# Autodesk Inventor assembly: Drivebase
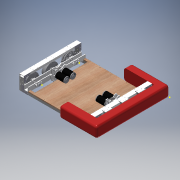
[picture p0: Inventor's stored thumbnail of the model, 180x180]
Saved by Autodesk Inventor 2019 (Build 230136000, 136)
## iProperties
Created: 2018-06-29
Part Number: Drivebase
Document SubType Name: Assembly
Designer: s-2512711
Author: s-2512711
## Documents named in this file (17)
- D:\Summer Drive Base V1\Summer Drivebase\Summer Drivebase.iam
- D:\Summer Drive Base V1\Summer Drivebase\1x1.ipt
- D:\Summer Drive Base V1\Summer Drivebase\pan.ipt
- D:\Summer Drive Base V1\Summer Drivebase\Drivebase PowerUp Files\Gearbox.iam
- D:\Summer Drive Base V1\Summer Drivebase\U.ipt
- D:\Summer Drive Base V1\Summer Drivebase\Drivebase PowerUp Files\Gearbox_CPY.iam
- D:\Summer Drive Base V1\Summer Drivebase\Drivebase PowerUp Files\4461-17-0101 + Bearing.iam
- D:\Summer Drive Base V1\Summer Drivebase\16th hex spacer.ipt
- D:\Summer Drive Base V1\Summer Drivebase\colsonwgeelwithhub.iam
- D:\Summer Drive Base V1\Summer Drivebase\475 hex shaft.ipt
- D:\Summer Drive Base V1\Summer Drivebase\am-1238+Collar+Clamp,+0.5''+Hex+Bore,+Aluminum.iam
- D:\Summer Drive Base V1\Summer Drivebase\Drivebase PowerUp Files\Omni Wheel.iam
- D:\Summer Drive Base V1\Summer Drivebase\525 hex shaft.ipt
- D:\Summer Drive Base V1\Summer Drivebase\5.5 2x2.ipt
- D:\Summer Drive Base V1\Summer Drivebase\26 1x2.ipt
- D:\Summer Drive Base V1\Summer Drivebase\L gusset.ipt
- D:\Summer Drive Base V1\Summer Drivebase\Bumper v2.iam
## Components (65 placed, 16 different names)
1. 1x1:1 — Mate:22, Mate:23, Mate:24, Mate:25, Mate:26, Mate:33, Mate:34, Mate:35, Mate:130, Mate:134
2. 1x1:2 — Mate:48, Mate:49, Mate:50, Mate:128, Mate:136, Mate:137, Mate:169, Mate:170
3. pan:1 — Mate:22, Mate:23, Mate:46, Mate:47
4. Gearbox:1 [sub-assembly] — Mate:36, Mate:37, Mate:42, Rotation:1, Mate:67, Mate:68, Mate:76, Mate:77
5. Gearbox:2 [sub-assembly] — Mate:38, Mate:39, Mate:40, Rotation:2, Mate:70, Mate:71, Mate:73, Mate:74
6. U:1 — Mate:33, Mate:34, Mate:35, Mate:38, Mate:39, Mate:40, Mate:44, Mate:45, Mate:46, Mate:47, Mate:48, Mate:49, Mate:50, Mate:51, Mate:52, Angle:1, Mate:53, Mate:54, Angle:2, Mate:55, Mate:56, Angle:3, Mate:57, Mate:58, Angle:4, Mate:132, Mate:133, Mate:135
7. U:2 — Mate:24, Mate:25, Mate:26, Mate:36, Mate:37, Mate:41, Mate:42, Mate:43, Mate:59, Mate:60, Angle:5, Mate:61, Mate:62, Angle:6, Mate:63, Mate:64, Angle:7, Mate:65, Mate:66, Angle:8, Mate:126, Mate:127, Mate:129, Mate:131, Mate:179
8. Gearbox_CPY:1 [sub-assembly] — Mate:44, Mate:45, Rotation:2, Mate:72
9. Gearbox_CPY:2 [sub-assembly] — Mate:41, Mate:43, Rotation:1, Mate:69
10. 4461-17-0101 + Bearing:1 [sub-assembly] — Mate:55, Mate:56, Angle:3, Mate:98
11. 4461-17-0101 + Bearing:2 [sub-assembly] — Mate:51, Mate:52, Angle:1, Mate:118
12. 4461-17-0101 + Bearing:3 [sub-assembly] — Mate:63, Mate:64, Angle:7, Mate:104, Flush:6, Flush:7
13. 4461-17-0101 + Bearing:4 [sub-assembly] — Mate:59, Mate:60, Angle:5, Mate:79, Mate:80, Mate:81, Rotation:3
14. 4461-17-0101 + Bearing:5 [sub-assembly] — Mate:61, Mate:62, Angle:6, Mate:86
15. 4461-17-0101 + Bearing:6 [sub-assembly] — Mate:65, Mate:66, Angle:8, Mate:109
16. 4461-17-0101 + Bearing:7 [sub-assembly] — Mate:53, Mate:54, Angle:2, Mate:115, Flush:10, Flush:11
17. 4461-17-0101 + Bearing:8 [sub-assembly] — Mate:57, Mate:58, Angle:4, Mate:92, Mate:93, Flush:3
18. 16th hex spacer:1 — Mate:67, Mate:68, Mate:69, Mate:78
19. 16th hex spacer:2 — Mate:70, Mate:71, Mate:72, Mate:75
20. colsonwgeelwithhub:1 [sub-assembly] — Mate:73, Mate:74, Mate:75
21. colsonwgeelwithhub:2 [sub-assembly] — Mate:76, Mate:77, Mate:78
22. 475 hex shaft:1 — Flush:4, Mate:94, Mate:95, Mate:96, Mate:97, Mate:100, Mate:101, Flush:5, Mate:102, Mate:103
23. 475 hex shaft:2 — Mate:82, Mate:83, Flush:1, Mate:84, Mate:85, Mate:87, Mate:88, Mate:90, Mate:91, Flush:2
24. am-1238+Collar+Clamp,+0.5''+Hex+Bore,+Aluminum:1 [sub-assembly] — Mate:92, Mate:93, Flush:3, Flush:4, Mate:94, Mate:95
25. am-1238+Collar+Clamp,+0.5''+Hex+Bore,+Aluminum:2 [sub-assembly] — Mate:79, Mate:80, Mate:81, Rotation:3, Mate:82, Mate:83, Flush:1
26. am-1238+Collar+Clamp,+0.5''+Hex+Bore,+Aluminum:3 [sub-assembly] — Mate:90, Mate:91, Flush:2
27. am-1238+Collar+Clamp,+0.5''+Hex+Bore,+Aluminum:4 [sub-assembly] — Flush:5, Mate:102, Mate:103
28. Omni Wheel:1 [sub-assembly] — Mate:87, Mate:88, Mate:89
29. Omni Wheel:2 [sub-assembly] — Mate:99, Mate:100, Mate:101
30. 16th hex spacer:3 — Mate:84, Mate:85, Mate:86, Mate:89
31. 16th hex spacer:4 — Mate:96, Mate:97, Mate:98, Mate:99
32. 525 hex shaft:1 — Flush:12, Mate:116, Mate:117, Mate:119, Mate:120, Mate:122, Mate:123, Flush:13, Mate:124, Mate:125
33. 525 hex shaft:2 — Flush:8, Mate:105, Mate:106, Mate:107, Mate:108, Mate:110, Mate:111, Mate:113, Mate:114, Flush:9
34. am-1238+Collar+Clamp,+0.5''+Hex+Bore,+Aluminum:5 [sub-assembly] — Mate:115, Flush:10, Flush:11, Flush:12, Mate:116, Mate:117
35. am-1238+Collar+Clamp,+0.5''+Hex+Bore,+Aluminum:6 [sub-assembly] — Mate:104, Flush:6, Flush:7, Flush:8, Mate:105, Mate:106
36. am-1238+Collar+Clamp,+0.5''+Hex+Bore,+Aluminum:7 [sub-assembly] — Flush:13, Mate:124, Mate:125
37. am-1238+Collar+Clamp,+0.5''+Hex+Bore,+Aluminum:8 [sub-assembly] — Mate:113, Mate:114, Flush:9
38. colsonwgeelwithhub:3 [sub-assembly] — Mate:110, Mate:111, Mate:112
39. colsonwgeelwithhub:4 [sub-assembly] — Mate:121, Mate:122, Mate:123
40. 16th hex spacer:5 — Mate:107, Mate:108, Mate:109, Mate:112
41. 16th hex spacer:6 — Mate:118, Mate:119, Mate:120, Mate:121
42. 5.5 2x2:1 — Mate:126, Mate:127, Mate:128, Mate:138, Mate:139, Mate:140, Mate:148, Mate:168, Mate:171, Mate:172, Mate:196
43. 5.5 2x2:2 — Mate:135, Mate:136, Mate:137, Mate:141, Mate:142, Mate:143, Mate:152, Mate:155, Mate:186, Mate:188, Mate:189, Mate:190, Mate:191, Mate:192
44. 5.5 2x2:3 — Mate:132, Mate:133, Mate:134, Mate:180, Mate:182, Mate:183, Mate:184, Mate:193, Mate:194, Mate:198
45. 5.5 2x2:4 — Mate:129, Mate:130, Mate:131, Mate:174, Mate:176, Mate:177, Mate:178, Mate:195
46. 26 1x2:1 — Mate:141, Mate:142, Mate:143, Mate:150, Mate:151, Mate:153, Mate:154, Mate:156, Mate:157, Mate:158, Mate:159, Mate:160, Mate:161, Mate:197, Mate:199
47. 26 1x2:2 — Mate:138, Mate:139, Mate:140, Mate:144, Mate:145, Mate:146, Mate:147, Mate:149, Mate:162, Mate:163, Mate:164, Mate:165, Mate:166, Mate:167, Mate:200, Mate:201, Mate:202
48. L gusset:1 — Mate:153, Mate:154, Mate:155
49. L gusset:2 — Mate:150, Mate:151, Mate:152
50. L gusset:3 — Mate:159, Mate:160, Mate:161
51. L gusset:4 — Mate:156, Mate:157, Mate:158
52. L gusset:5 — Mate:162, Mate:163, Mate:164
53. L gusset:6 — Mate:165, Mate:166, Mate:167
54. L gusset:7 — Mate:147, Mate:148, Mate:149
55. L gusset:8 — Mate:144, Mate:145, Mate:146
56. L gusset:9 — Mate:189, Mate:190, Mate:191
57. L gusset:10 — Mate:186, Mate:188, Mate:192
58. L gusset:11 — Mate:183, Mate:184, Mate:194
59. L gusset:12 — Mate:180, Mate:182, Mate:193
60. L gusset:13 — Mate:174, Mate:176, Mate:195
61. L gusset:14 — Mate:177, Mate:178, Mate:179
62. L gusset:15 — Mate:171, Mate:172, Mate:196
63. L gusset:16 — Mate:168, Mate:169, Mate:170
64. Bumper v2:1 [sub-assembly] — Mate:200, Mate:201, Mate:202
65. Bumper v2:2 [sub-assembly] — Mate:197, Mate:198, Mate:199
## Relationships (194: Mate 170, Flush 13, Angle 8, RelateRotation 3)
- Mate:22: 1x1:1 ↔ pan:1
- Mate:23: 1x1:1 ↔ pan:1
- Mate:24: 1x1:1 ↔ U:2
- Mate:25: 1x1:1 ↔ U:2
- Mate:26: 1x1:1 ↔ U:2
- Mate:33: 1x1:1 ↔ U:1
- Mate:34: 1x1:1 ↔ U:1
- Mate:35: 1x1:1 ↔ U:1
- Mate:36: Gearbox:1 ↔ U:2
- Mate:37: Gearbox:1 ↔ U:2
- Mate:38: Gearbox:2 ↔ U:1
- Mate:39: Gearbox:2 ↔ U:1
- Mate:40: Gearbox:2 ↔ U:1
- Mate:41: U:2 ↔ Gearbox_CPY:2
- Mate:42: Gearbox:1 ↔ U:2
- Mate:43: U:2 ↔ Gearbox_CPY:2
- Rotation:1 [RelateRotation] (1 ul): Gearbox:1 ↔ Gearbox_CPY:2
- Mate:44: U:1 ↔ Gearbox_CPY:1
- Mate:45: U:1 ↔ Gearbox_CPY:1
- Rotation:2 [RelateRotation] (1 ul): Gearbox:2 ↔ Gearbox_CPY:1
- Mate:46: pan:1 ↔ U:1
- Mate:47: pan:1 ↔ U:1
- Mate:48: 1x1:2 ↔ U:1
- Mate:49: 1x1:2 ↔ U:1
- Mate:50: 1x1:2 ↔ U:1
- Mate:51: U:1 ↔ 4461-17-0101 + Bearing:2
- Mate:52: U:1 ↔ 4461-17-0101 + Bearing:2
- Angle:1 (0 deg): U:1 ↔ 4461-17-0101 + Bearing:2
- Mate:53: U:1 ↔ 4461-17-0101 + Bearing:7
- Mate:54: U:1 ↔ 4461-17-0101 + Bearing:7
- Angle:2 (0 deg): U:1 ↔ 4461-17-0101 + Bearing:7
- Mate:55: U:1 ↔ 4461-17-0101 + Bearing:1
- Mate:56: U:1 ↔ 4461-17-0101 + Bearing:1
- Angle:3 (0 deg): U:1 ↔ 4461-17-0101 + Bearing:1
- Mate:57: U:1 ↔ 4461-17-0101 + Bearing:8
- Mate:58: U:1 ↔ 4461-17-0101 + Bearing:8
- Angle:4 (0 deg): U:1 ↔ 4461-17-0101 + Bearing:8
- Mate:59: U:2 ↔ 4461-17-0101 + Bearing:4
- Mate:60: U:2 ↔ 4461-17-0101 + Bearing:4
- Angle:5 (0 deg): U:2 ↔ 4461-17-0101 + Bearing:4
- Mate:61: U:2 ↔ 4461-17-0101 + Bearing:5
- Mate:62: U:2 ↔ 4461-17-0101 + Bearing:5
- Angle:6 (0 deg): U:2 ↔ 4461-17-0101 + Bearing:5
- Mate:63: U:2 ↔ 4461-17-0101 + Bearing:3
- Mate:64: U:2 ↔ 4461-17-0101 + Bearing:3
- Angle:7 (0 deg): U:2 ↔ 4461-17-0101 + Bearing:3
- Mate:65: U:2 ↔ 4461-17-0101 + Bearing:6
- Mate:66: U:2 ↔ 4461-17-0101 + Bearing:6
- Angle:8 (0 deg): U:2 ↔ 4461-17-0101 + Bearing:6
- Mate:67: Gearbox:1 ↔ 16th hex spacer:1
- Mate:68: Gearbox:1 ↔ 16th hex spacer:1
- Mate:69: Gearbox_CPY:2 ↔ 16th hex spacer:1
- Mate:70: Gearbox:2 ↔ 16th hex spacer:2
- Mate:71: Gearbox:2 ↔ 16th hex spacer:2
- Mate:72: Gearbox_CPY:1 ↔ 16th hex spacer:2
- Mate:73: Gearbox:2 ↔ colsonwgeelwithhub:1
- Mate:74: Gearbox:2 ↔ colsonwgeelwithhub:1
- Mate:75: 16th hex spacer:2 ↔ colsonwgeelwithhub:1
- Mate:76: Gearbox:1 ↔ colsonwgeelwithhub:2
- Mate:77: Gearbox:1 ↔ colsonwgeelwithhub:2
- Mate:78: 16th hex spacer:1 ↔ colsonwgeelwithhub:2
- Mate:79: 4461-17-0101 + Bearing:4 ↔ am-1238+Collar+Clamp,+0.5''+Hex+Bore,+Aluminum:2
- Mate:80: 4461-17-0101 + Bearing:4 ↔ am-1238+Collar+Clamp,+0.5''+Hex+Bore,+Aluminum:2
- Mate:81: 4461-17-0101 + Bearing:4 ↔ am-1238+Collar+Clamp,+0.5''+Hex+Bore,+Aluminum:2
- Rotation:3 [RelateRotation] (1 ul): 4461-17-0101 + Bearing:4 ↔ am-1238+Collar+Clamp,+0.5''+Hex+Bore,+Aluminum:2
- Mate:82: 475 hex shaft:2 ↔ am-1238+Collar+Clamp,+0.5''+Hex+Bore,+Aluminum:2
- Mate:83: 475 hex shaft:2 ↔ am-1238+Collar+Clamp,+0.5''+Hex+Bore,+Aluminum:2
- Flush:1: 475 hex shaft:2 ↔ am-1238+Collar+Clamp,+0.5''+Hex+Bore,+Aluminum:2
- Mate:84: 475 hex shaft:2 ↔ 16th hex spacer:3
- Mate:85: 475 hex shaft:2 ↔ 16th hex spacer:3
- Mate:86: 4461-17-0101 + Bearing:5 ↔ 16th hex spacer:3
- Mate:87: 475 hex shaft:2 ↔ Omni Wheel:1
- Mate:88: 475 hex shaft:2 ↔ Omni Wheel:1
- Mate:89: Omni Wheel:1 ↔ 16th hex spacer:3
- Mate:90: 475 hex shaft:2 ↔ am-1238+Collar+Clamp,+0.5''+Hex+Bore,+Aluminum:3
- Mate:91: 475 hex shaft:2 ↔ am-1238+Collar+Clamp,+0.5''+Hex+Bore,+Aluminum:3
- Flush:2: 475 hex shaft:2 ↔ am-1238+Collar+Clamp,+0.5''+Hex+Bore,+Aluminum:3
- Mate:92: 4461-17-0101 + Bearing:8 ↔ am-1238+Collar+Clamp,+0.5''+Hex+Bore,+Aluminum:1
- Mate:93: 4461-17-0101 + Bearing:8 ↔ am-1238+Collar+Clamp,+0.5''+Hex+Bore,+Aluminum:1
- Flush:3: 4461-17-0101 + Bearing:8 ↔ am-1238+Collar+Clamp,+0.5''+Hex+Bore,+Aluminum:1
- Flush:4: 475 hex shaft:1 ↔ am-1238+Collar+Clamp,+0.5''+Hex+Bore,+Aluminum:1
- Mate:94: 475 hex shaft:1 ↔ am-1238+Collar+Clamp,+0.5''+Hex+Bore,+Aluminum:1
- Mate:95: 475 hex shaft:1 ↔ am-1238+Collar+Clamp,+0.5''+Hex+Bore,+Aluminum:1
- Mate:96: 475 hex shaft:1 ↔ 16th hex spacer:4
- Mate:97: 475 hex shaft:1 ↔ 16th hex spacer:4
- Mate:98: 4461-17-0101 + Bearing:1 ↔ 16th hex spacer:4
- Mate:99: Omni Wheel:2 ↔ 16th hex spacer:4
- Mate:100: 475 hex shaft:1 ↔ Omni Wheel:2
- Mate:101: 475 hex shaft:1 ↔ Omni Wheel:2
- Flush:5: 475 hex shaft:1 ↔ am-1238+Collar+Clamp,+0.5''+Hex+Bore,+Aluminum:4
- Mate:102: 475 hex shaft:1 ↔ am-1238+Collar+Clamp,+0.5''+Hex+Bore,+Aluminum:4
- Mate:103: 475 hex shaft:1 ↔ am-1238+Collar+Clamp,+0.5''+Hex+Bore,+Aluminum:4
- Mate:104: 4461-17-0101 + Bearing:3 ↔ am-1238+Collar+Clamp,+0.5''+Hex+Bore,+Aluminum:6
- Flush:6: 4461-17-0101 + Bearing:3 ↔ am-1238+Collar+Clamp,+0.5''+Hex+Bore,+Aluminum:6
- Flush:7: 4461-17-0101 + Bearing:3 ↔ am-1238+Collar+Clamp,+0.5''+Hex+Bore,+Aluminum:6
- Flush:8: 525 hex shaft:2 ↔ am-1238+Collar+Clamp,+0.5''+Hex+Bore,+Aluminum:6
- Mate:105: 525 hex shaft:2 ↔ am-1238+Collar+Clamp,+0.5''+Hex+Bore,+Aluminum:6
- Mate:106: 525 hex shaft:2 ↔ am-1238+Collar+Clamp,+0.5''+Hex+Bore,+Aluminum:6
- Mate:107: 525 hex shaft:2 ↔ 16th hex spacer:5
- Mate:108: 525 hex shaft:2 ↔ 16th hex spacer:5
- Mate:109: 4461-17-0101 + Bearing:6 ↔ 16th hex spacer:5
- Mate:110: 525 hex shaft:2 ↔ colsonwgeelwithhub:3
- Mate:111: 525 hex shaft:2 ↔ colsonwgeelwithhub:3
- Mate:112: colsonwgeelwithhub:3 ↔ 16th hex spacer:5
- Mate:113: 525 hex shaft:2 ↔ am-1238+Collar+Clamp,+0.5''+Hex+Bore,+Aluminum:8
- Mate:114: 525 hex shaft:2 ↔ am-1238+Collar+Clamp,+0.5''+Hex+Bore,+Aluminum:8
- Flush:9: 525 hex shaft:2 ↔ am-1238+Collar+Clamp,+0.5''+Hex+Bore,+Aluminum:8
- Mate:115: 4461-17-0101 + Bearing:7 ↔ am-1238+Collar+Clamp,+0.5''+Hex+Bore,+Aluminum:5
- Flush:10: 4461-17-0101 + Bearing:7 ↔ am-1238+Collar+Clamp,+0.5''+Hex+Bore,+Aluminum:5
- Flush:11: 4461-17-0101 + Bearing:7 ↔ am-1238+Collar+Clamp,+0.5''+Hex+Bore,+Aluminum:5
- Flush:12: 525 hex shaft:1 ↔ am-1238+Collar+Clamp,+0.5''+Hex+Bore,+Aluminum:5
- Mate:116: 525 hex shaft:1 ↔ am-1238+Collar+Clamp,+0.5''+Hex+Bore,+Aluminum:5
- Mate:117: 525 hex shaft:1 ↔ am-1238+Collar+Clamp,+0.5''+Hex+Bore,+Aluminum:5
- Mate:118: 4461-17-0101 + Bearing:2 ↔ 16th hex spacer:6
- Mate:119: 525 hex shaft:1 ↔ 16th hex spacer:6
- Mate:120: 525 hex shaft:1 ↔ 16th hex spacer:6
- Mate:121: colsonwgeelwithhub:4 ↔ 16th hex spacer:6
- Mate:122: 525 hex shaft:1 ↔ colsonwgeelwithhub:4
- Mate:123: 525 hex shaft:1 ↔ colsonwgeelwithhub:4
- Flush:13: 525 hex shaft:1 ↔ am-1238+Collar+Clamp,+0.5''+Hex+Bore,+Aluminum:7
- Mate:124: 525 hex shaft:1 ↔ am-1238+Collar+Clamp,+0.5''+Hex+Bore,+Aluminum:7
- Mate:125: 525 hex shaft:1 ↔ am-1238+Collar+Clamp,+0.5''+Hex+Bore,+Aluminum:7
- Mate:126: U:2 ↔ 5.5 2x2:1
- Mate:127: U:2 ↔ 5.5 2x2:1
- Mate:128: 1x1:2 ↔ 5.5 2x2:1
- Mate:129: U:2 ↔ 5.5 2x2:4
- Mate:130: 1x1:1 ↔ 5.5 2x2:4
- Mate:131: U:2 ↔ 5.5 2x2:4
- Mate:132: U:1 ↔ 5.5 2x2:3
- Mate:133: U:1 ↔ 5.5 2x2:3
- Mate:134: 1x1:1 ↔ 5.5 2x2:3
- Mate:135: U:1 ↔ 5.5 2x2:2
- Mate:136: 1x1:2 ↔ 5.5 2x2:2
- Mate:137: 1x1:2 ↔ 5.5 2x2:2
- Mate:138: 5.5 2x2:1 ↔ 26 1x2:2
- Mate:139: 5.5 2x2:1 ↔ 26 1x2:2
- Mate:140: 5.5 2x2:1 ↔ 26 1x2:2
- Mate:141: 5.5 2x2:2 ↔ 26 1x2:1
- Mate:142: 5.5 2x2:2 ↔ 26 1x2:1
- Mate:143: 5.5 2x2:2 ↔ 26 1x2:1
- Mate:144: 26 1x2:2 ↔ L gusset:8
- Mate:145: 26 1x2:2 ↔ L gusset:8
- Mate:146: 26 1x2:2 ↔ L gusset:8
- Mate:147: 26 1x2:2 ↔ L gusset:7
- Mate:148: 5.5 2x2:1 ↔ L gusset:7
- Mate:149: 26 1x2:2 ↔ L gusset:7
- Mate:150: 26 1x2:1 ↔ L gusset:2
- Mate:151: 26 1x2:1 ↔ L gusset:2
- Mate:152: 5.5 2x2:2 ↔ L gusset:2
- Mate:153: 26 1x2:1 ↔ L gusset:1
- Mate:154: 26 1x2:1 ↔ L gusset:1
- Mate:155: 5.5 2x2:2 ↔ L gusset:1
- Mate:156: 26 1x2:1 ↔ L gusset:4
- Mate:157: 26 1x2:1 ↔ L gusset:4
- Mate:158: 26 1x2:1 ↔ L gusset:4
- Mate:159: 26 1x2:1 ↔ L gusset:3
- Mate:160: 26 1x2:1 ↔ L gusset:3
- Mate:161: 26 1x2:1 ↔ L gusset:3
- Mate:162: 26 1x2:2 ↔ L gusset:5
- Mate:163: 26 1x2:2 ↔ L gusset:5
- Mate:164: 26 1x2:2 ↔ L gusset:5
- Mate:165: 26 1x2:2 ↔ L gusset:6
- Mate:166: 26 1x2:2 ↔ L gusset:6
- Mate:167: 26 1x2:2 ↔ L gusset:6
- Mate:168: 5.5 2x2:1 ↔ L gusset:16
- Mate:169: 1x1:2 ↔ L gusset:16
- Mate:170: 1x1:2 ↔ L gusset:16
- Mate:171: 5.5 2x2:1 ↔ L gusset:15
- Mate:172: 5.5 2x2:1 ↔ L gusset:15
- Mate:174: 5.5 2x2:4 ↔ L gusset:13
- Mate:176: 5.5 2x2:4 ↔ L gusset:13
- Mate:177: 5.5 2x2:4 ↔ L gusset:14
- Mate:178: 5.5 2x2:4 ↔ L gusset:14
- Mate:179: U:2 ↔ L gusset:14
- Mate:180: 5.5 2x2:3 ↔ L gusset:12
- Mate:182: 5.5 2x2:3 ↔ L gusset:12
- Mate:183: 5.5 2x2:3 ↔ L gusset:11
- Mate:184: 5.5 2x2:3 ↔ L gusset:11
- Mate:186: 5.5 2x2:2 ↔ L gusset:10
- Mate:188: 5.5 2x2:2 ↔ L gusset:10
- Mate:189: 5.5 2x2:2 ↔ L gusset:9
- Mate:190: 5.5 2x2:2 ↔ L gusset:9
- Mate:191: 5.5 2x2:2 ↔ L gusset:9
- Mate:192: 5.5 2x2:2 ↔ L gusset:10
- Mate:193: 5.5 2x2:3 ↔ L gusset:12
- Mate:194: 5.5 2x2:3 ↔ L gusset:11
- Mate:195: 5.5 2x2:4 ↔ L gusset:13
- Mate:196: 5.5 2x2:1 ↔ L gusset:15
- Mate:197: 26 1x2:1 ↔ Bumper v2:2
- Mate:198: 5.5 2x2:3 ↔ Bumper v2:2
- Mate:199: 26 1x2:1 ↔ Bumper v2:2
- Mate:200: 26 1x2:2 ↔ Bumper v2:1
- Mate:201: 26 1x2:2 ↔ Bumper v2:1
- Mate:202: 26 1x2:2 ↔ Bumper v2:1
